# Autodesk Inventor assembly: battery_box_5V
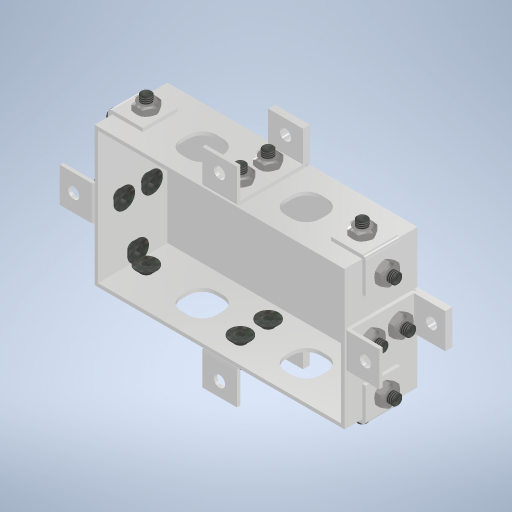
[picture p0: Inventor's stored thumbnail of the model, 512x512]
Saved by Autodesk Inventor 2023 (Build 270158000, 158)
## iProperties
Created: 2023-05-28
Part Number: battery_box_5V
Document SubType Name: Assembly
Designer: 310611102
Mass: 39.6762 g
Surface Area: 243.188 cm^2
Volume: 11.1195 cm^3
Density: 3.56818 g/cm^3
Author: 310611102
## Documents named in this file (8)
- C:\Users\310611102\Documents\Inventor\SSR\avionics_2023ver\electronics\battery box2\battery_box_5V_ver2\battery_box_5V.iam
- C:\Users\310611102\Documents\Inventor\SSR\avionics_2023ver\electronics\battery box2\battery_box_5V_ver2\battery_box_5V_base.ipt
- C:\Users\310611102\Documents\Inventor\SSR\avionics_2023ver\electronics\battery box2\battery_box_5V_ver2\battery_box_5V_side1.ipt
- C:\Users\310611102\Documents\Inventor\SSR\avionics_2023ver\electronics\battery box2\battery_box_5V_ver2\connector.ipt
- C:\Users\310611102\Documents\Inventor\SSR\avionics_2023ver\electronics\battery box2\battery_box_5V_ver2\battery_box_5V_front.ipt
- C:\Users\310611102\Documents\Inventor\SSR\avionics_2023ver\electronics\battery box2\battery_box_5V_ver2\battery_box_5V_back.ipt
- C:\Users\310611102\Documents\Inventor\Content Center Files\R2023\en-US\ISO 10642(1)\ISO 10642 - M3 x  8.ipt
- C:\Users\310611102\Documents\Inventor\Content Center Files\R2023\en-US\ISO 4032(2)\ISO 4032 - M3 - ISO.ipt
## Components (49 placed, 7 different names)
1. battery_box_5V_base:1 — Insert:1, Insert:3, Insert:15, Mate:2, Flush:2, Mate:3, Flush:5, Insert:43
2. battery_box_5V_side1:1 — Insert:42, Insert:46, Cylindrical:26, Cylindrical:28, Insert:58, Insert:59, Insert:60, Insert:61
3. connector:1 — Insert:1, Insert:42, Insert:74
4. connector:3 — Insert:3, Insert:44, Insert:68
5. connector:4 — Insert:46, Insert:75
6. battery_box_5V_side1:2 — Insert:44, Insert:47, Cylindrical:25, Cylindrical:30, Insert:50, Insert:51, Insert:52, Insert:53
7. battery_box_5V_front:1 — Mate:2, Flush:2, Insert:36, Cylindrical:23, Insert:45, Cylindrical:29, Insert:54, Insert:55, Insert:56, Insert:57
8. connector:5 — Insert:47, Insert:66
9. connector:6 — Cylindrical:22, Insert:43, Insert:71
10. connector:9 — Insert:45, Insert:79
11. connector:14 — Insert:15, Insert:36, Insert:78
12. connector:18 — Cylindrical:23, Cylindrical:28, Insert:76, Insert:77
13. battery_box_5V_back:1 — Mate:3, Cylindrical:22, Flush:5, Insert:48, Cylindrical:24, Cylindrical:27, Insert:62, Insert:63, Insert:64, Insert:65
14. connector:19 — Insert:48, Insert:70
15. connector:20 — Cylindrical:24, Cylindrical:25, Insert:67, Insert:69
16. connector:21 — Cylindrical:26, Cylindrical:27, Insert:72, Insert:73
17. connector:22 — Cylindrical:29, Cylindrical:30, Mate:5, Insert:80
18. ISO 10642 M3x8:1 — Mate:4, Insert:50
19. ISO 10642 M3x8:2 — Insert:51
20. ISO 10642 M3x8:3 — Insert:52
21. ISO 10642 M3x8:4 — Insert:53
22. ISO 10642 M3x8:5 — Insert:54
23. ISO 10642 M3x8:6 — Insert:55
24. ISO 10642 M3x8:7 — Insert:56
25. ISO 10642 M3x8:8 — Insert:57
26. ISO 10642 M3x8:9 — Insert:58
27. ISO 10642 M3x8:10 — Insert:59
28. ISO 10642 M3x8:11 — Insert:60
29. ISO 10642 M3x8:12 — Insert:61
30. ISO 10642 M3x8:13 — Insert:62
31. ISO 10642 M3x8:14 — Insert:63
32. ISO 10642 M3x8:15 — Insert:64
33. ISO 10642 M3x8:16 — Insert:65
34. ISO 4032 M3:1 — Mate:4, Mate:5
35. ISO 4032 M3:2 — Insert:66
36. ISO 4032 M3:3 — Insert:67
37. ISO 4032 M3:4 — Insert:68
38. ISO 4032 M3:5 — Insert:69
39. ISO 4032 M3:6 — Insert:70
40. ISO 4032 M3:7 — Insert:71
41. ISO 4032 M3:8 — Insert:72
42. ISO 4032 M3:9 — Insert:73
43. ISO 4032 M3:10 — Insert:74
44. ISO 4032 M3:11 — Insert:75
45. ISO 4032 M3:12 — Insert:76
46. ISO 4032 M3:13 — Insert:77
47. ISO 4032 M3:14 — Insert:78
48. ISO 4032 M3:15 — Insert:79
49. ISO 4032 M3:16 — Insert:80
## Relationships (57: Insert 42, CylindricalJoint 9, Mate 4, Flush 2)
- Insert:1: battery_box_5V_base:1 ↔ connector:1
- Insert:3: battery_box_5V_base:1 ↔ connector:3
- Insert:15: battery_box_5V_base:1 ↔ connector:14
- Mate:2: battery_box_5V_base:1 ↔ battery_box_5V_front:1
- Flush:2: battery_box_5V_base:1 ↔ battery_box_5V_front:1
- Insert:36: battery_box_5V_front:1 ↔ connector:14
- Mate:3: battery_box_5V_base:1 ↔ battery_box_5V_back:1
- Cylindrical:22: connector:6 ↔ battery_box_5V_back:1
- Flush:5: battery_box_5V_base:1 ↔ battery_box_5V_back:1
- Insert:42: battery_box_5V_side1:1 ↔ connector:1
- Insert:43: battery_box_5V_base:1 ↔ connector:6
- Insert:44: connector:3 ↔ battery_box_5V_side1:2
- Cylindrical:23: battery_box_5V_front:1 ↔ connector:18
- Insert:45: battery_box_5V_front:1 ↔ connector:9
- Insert:46: battery_box_5V_side1:1 ↔ connector:4
- Insert:47: battery_box_5V_side1:2 ↔ connector:5
- Insert:48: battery_box_5V_back:1 ↔ connector:19
- Cylindrical:24: battery_box_5V_back:1 ↔ connector:20
- Cylindrical:25: battery_box_5V_side1:2 ↔ connector:20
- Cylindrical:26: battery_box_5V_side1:1 ↔ connector:21
- Cylindrical:27: battery_box_5V_back:1 ↔ connector:21
- Cylindrical:28: battery_box_5V_side1:1 ↔ connector:18
- Cylindrical:29: battery_box_5V_front:1 ↔ connector:22
- Cylindrical:30: battery_box_5V_side1:2 ↔ connector:22
- Mate:4: ISO 10642 M3x8:1 ↔ ISO 4032 M3:1
- Insert:50: battery_box_5V_side1:2 ↔ ISO 10642 M3x8:1
- Mate:5: connector:22 ↔ ISO 4032 M3:1
- Insert:51: battery_box_5V_side1:2 ↔ ISO 10642 M3x8:2
- Insert:52: battery_box_5V_side1:2 ↔ ISO 10642 M3x8:3
- Insert:53: battery_box_5V_side1:2 ↔ ISO 10642 M3x8:4
- Insert:54: battery_box_5V_front:1 ↔ ISO 10642 M3x8:5
- Insert:55: battery_box_5V_front:1 ↔ ISO 10642 M3x8:6
- Insert:56: battery_box_5V_front:1 ↔ ISO 10642 M3x8:7
- Insert:57: battery_box_5V_front:1 ↔ ISO 10642 M3x8:8
- Insert:58: battery_box_5V_side1:1 ↔ ISO 10642 M3x8:9
- Insert:59: battery_box_5V_side1:1 ↔ ISO 10642 M3x8:10
- Insert:60: battery_box_5V_side1:1 ↔ ISO 10642 M3x8:11
- Insert:61: battery_box_5V_side1:1 ↔ ISO 10642 M3x8:12
- Insert:62: battery_box_5V_back:1 ↔ ISO 10642 M3x8:13
- Insert:63: battery_box_5V_back:1 ↔ ISO 10642 M3x8:14
- Insert:64: battery_box_5V_back:1 ↔ ISO 10642 M3x8:15
- Insert:65: battery_box_5V_back:1 ↔ ISO 10642 M3x8:16
- Insert:66: connector:5 ↔ ISO 4032 M3:2
- Insert:67: connector:20 ↔ ISO 4032 M3:3
- Insert:68: connector:3 ↔ ISO 4032 M3:4
- Insert:69: connector:20 ↔ ISO 4032 M3:5
- Insert:70: connector:19 ↔ ISO 4032 M3:6
- Insert:71: connector:6 ↔ ISO 4032 M3:7
- Insert:72: connector:21 ↔ ISO 4032 M3:8
- Insert:73: connector:21 ↔ ISO 4032 M3:9
- Insert:74: connector:1 ↔ ISO 4032 M3:10
- Insert:75: connector:4 ↔ ISO 4032 M3:11
- Insert:76: connector:18 ↔ ISO 4032 M3:12
- Insert:77: connector:18 ↔ ISO 4032 M3:13
- Insert:78: connector:14 ↔ ISO 4032 M3:14
- Insert:79: connector:9 ↔ ISO 4032 M3:15
- Insert:80: connector:22 ↔ ISO 4032 M3:16
